# Autodesk Inventor assembly: Outer
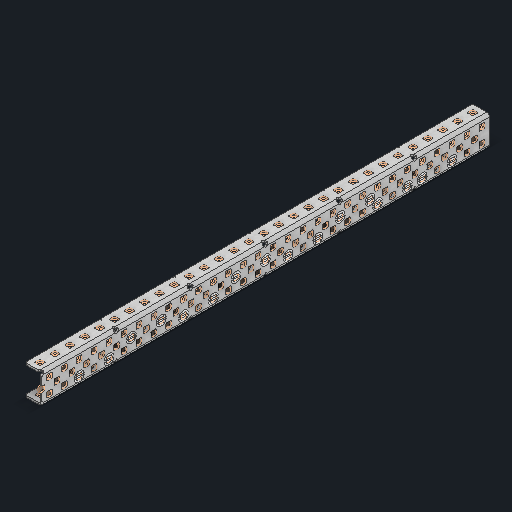
[picture p0: Inventor's stored thumbnail of the model, 512x512]
Saved by Autodesk Inventor 2025.1 (Build 291241000, 241)
## iProperties
Created: 2024-11-01
Part Number: Outer
Document SubType Name: Assembly
Designer: avere
Author: avere
## Documents named in this file (3)
- C:\Users\avere\VEX\High Stakes\CAD\V2\Chassis V2\Drivebay Left\Outer.iam
- C:\Users\avere\VEX\High Stakes\CAD\ROBOPROS-CAD-Inventor\Structure\C Channel\Aluminum 1x2x1\Alu C 1x2x1x30.ipt
- C:\Users\avere\VEX\High Stakes\CAD\ROBOPROS-CAD-Inventor\Quick Assemblies\Bearing Flat NScrew Slotted.iam
## Components (9 placed, 2 different names)
1. Alu C 1x2x1x30:1 — Mate:1, Flush:3, Flush:4, Insert:1, Mate:2, Insert:2, Mate:3, Insert:3, Mate:4, Insert:4, Mate:5
2. Bearing Flat NScrew Slotted:1 [sub-assembly] — Insert:1, Mate:2
3. Bearing Flat NScrew Slotted:2 [sub-assembly] — Insert:2, Mate:3
4. Bearing Flat NScrew Slotted:3 [sub-assembly] — Insert:3, Mate:4
5. Bearing Flat NScrew Slotted:4 [sub-assembly]
6. Bearing Flat NScrew Slotted:5 [sub-assembly]
7. Bearing Flat NScrew Slotted:6 [sub-assembly] — Insert:4, Mate:5
8. Bearing Flat NScrew Slotted:7 [sub-assembly]
9. Bearing Flat NScrew Slotted:8 [sub-assembly]
## Component patterns: (3 elements, first: Bearing Flat NScrew Slotted:3), (3 elements, first: Bearing Flat NScrew Slotted:6)
## Relationships (11: Mate 5, Insert 4, Flush 2)
- Mate:1 (-190.5 mm): Alu C 1x2x1x30:1
- Flush:3 (-12.7 mm): Alu C 1x2x1x30:1
- Flush:4 (-7.9375 mm): Alu C 1x2x1x30:1
- Insert:1: Alu C 1x2x1x30:1 ↔ Bearing Flat NScrew Slotted:1
- Mate:2: Alu C 1x2x1x30:1 ↔ Bearing Flat NScrew Slotted:1
- Insert:2: Alu C 1x2x1x30:1 ↔ Bearing Flat NScrew Slotted:2
- Mate:3: Alu C 1x2x1x30:1 ↔ Bearing Flat NScrew Slotted:2
- Insert:3: Alu C 1x2x1x30:1 ↔ Bearing Flat NScrew Slotted:3
- Mate:4: Alu C 1x2x1x30:1 ↔ Bearing Flat NScrew Slotted:3
- Insert:4: Alu C 1x2x1x30:1 ↔ Bearing Flat NScrew Slotted:6
- Mate:5: Alu C 1x2x1x30:1 ↔ Bearing Flat NScrew Slotted:6
